# Autodesk Inventor assembly: Leg_joint_roll_yaw
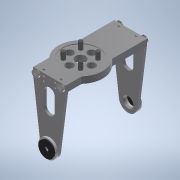
[picture p0: Inventor's stored thumbnail of the model, 180x180]
Saved by Autodesk Inventor 2020.4 (Build 244396000, 396)
## iProperties
Created: 2016-05-01
Part Number: Leg_joint_roll_yaw
Document SubType Name: Assembly
Designer: hiroaki
Mass: 101.489 g
Surface Area: 218.083 cm^2
Volume: 17.9148 cm^3
Density: 5.6651 g/cm^3
Author: hiroaki
## Documents named in this file (7)
- C:\Users\Masato\Documents\Inventor\CIT Brains_Inventor\OpenPlatform_ver3_0（ワッシャ変更）\LowerBody\Leg_joit\Leg_joint_roll_yaw.iam
- C:\Users\Masato\Documents\Inventor\CIT Brains_Inventor\OpenPlatform_ver3_0（ワッシャ変更）\LowerBody\Leg_joit\Leg_joint_slider_frame.ipt
- C:\Users\Masato\Documents\Inventor\CIT Brains_Inventor\OpenPlatform_ver3_0（ワッシャ変更）\Ready_Made\UUW-0312-10BH.ipt
- C:\Users\Masato\Documents\Inventor\CIT Brains_Inventor\OpenPlatform_ver3_0（ワッシャ変更）\LowerBody\Leg_joit\Leg_joint_yaw_frame.ipt
- C:\Users\Masato\Documents\Inventor\CIT Brains_Inventor\OpenPlatform_ver3_0（ワッシャ変更）\Ready_Made\Screw\M3-10.ipt
- C:\Users\Masato\Documents\Inventor\CIT Brains_Inventor\OpenPlatform_ver3_0（ワッシャ変更）\Ready_Made\Screw\M3-6.ipt
- C:\Users\Masato\Documents\Inventor\CIT Brains_Inventor\OpenPlatform_ver3_0（ワッシャ変更）\Ready_Made\TT-0814-15.ipt
## Components (15 placed, 6 different names)
1. Leg_joint_slider_frame:1 — 挿入:51, 挿入:52, 挿入:59, 挿入:60, 挿入:61
2. Leg_joint_slider_frame:2 — 挿入:49, 挿入:50, 挿入:57, 挿入:58, 挿入:62
3. UUW-0312-10BH:3 — 挿入:63
4. UUW-0312-10BH:4 — 挿入:64
5. Leg_joint_yaw_frame:1 — 挿入:49, 挿入:50, 挿入:51, 挿入:52, 挿入:53, 挿入:54, 挿入:55, 挿入:56
6. M3-10:1 — 挿入:53
7. M3-10:2 — 挿入:54
8. M3-10:3 — 挿入:55
9. M3-10:4 — 挿入:56
10. M3-6:1 — 挿入:57
11. M3-6:2 — 挿入:58
12. M3-6:3 — 挿入:59
13. M3-6:4 — 挿入:60
14. TT-0814-15:1 — 挿入:61, 挿入:64
15. TT-0814-15:2 — 挿入:62, 挿入:63
## Relationships (16: Insert 16)
- 挿入:49 [Insert]: Leg_joint_slider_frame:2 ↔ Leg_joint_yaw_frame:1
- 挿入:50 [Insert]: Leg_joint_slider_frame:2 ↔ Leg_joint_yaw_frame:1
- 挿入:51 [Insert]: Leg_joint_slider_frame:1 ↔ Leg_joint_yaw_frame:1
- 挿入:52 [Insert]: Leg_joint_slider_frame:1 ↔ Leg_joint_yaw_frame:1
- 挿入:53 [Insert]: Leg_joint_yaw_frame:1 ↔ M3-10:1
- 挿入:54 [Insert]: Leg_joint_yaw_frame:1 ↔ M3-10:2
- 挿入:55 [Insert]: Leg_joint_yaw_frame:1 ↔ M3-10:3
- 挿入:56 [Insert]: Leg_joint_yaw_frame:1 ↔ M3-10:4
- 挿入:57 [Insert]: Leg_joint_slider_frame:2 ↔ M3-6:1
- 挿入:58 [Insert]: Leg_joint_slider_frame:2 ↔ M3-6:2
- 挿入:59 [Insert]: Leg_joint_slider_frame:1 ↔ M3-6:3
- 挿入:60 [Insert]: Leg_joint_slider_frame:1 ↔ M3-6:4
- 挿入:61 [Insert]: Leg_joint_slider_frame:1 ↔ TT-0814-15:1
- 挿入:62 [Insert]: Leg_joint_slider_frame:2 ↔ TT-0814-15:2
- 挿入:63 [Insert]: UUW-0312-10BH:3 ↔ TT-0814-15:2
- 挿入:64 [Insert]: UUW-0312-10BH:4 ↔ TT-0814-15:1
